# Autodesk Inventor assembly: 机械架构
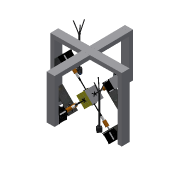
[picture p0: Inventor's stored thumbnail of the model, 180x180]
Saved by Autodesk Inventor 2016 (Build 200138000, 138)
## iProperties
Created: 2019-05-19
Part Number: 机械架构
Material: 常规
Document SubType Name: Assembly
Designer: oldboy
Author: oldboy
## Documents named in this file (14)
- F:\folder\毕业设计\解魔方机器人\机械结构\机械架构.iam
- F:\folder\毕业设计\解魔方机器人\机械结构\步进电机.ipt
- F:\folder\毕业设计\解魔方机器人\机械结构\杆件.ipt
- F:\folder\毕业设计\解魔方机器人\机械结构\联轴器.ipt
- F:\folder\毕业设计\解魔方机器人\机械结构\机械爪六角筒.ipt
- F:\folder\毕业设计\解魔方机器人\机械结构\机械架构\设计加速器\压缩弹簧1.iam
- F:\folder\毕业设计\解魔方机器人\机械结构\螺母.ipt
- F:\folder\毕业设计\解魔方机器人\机械结构\欧标铝.ipt
- F:\folder\毕业设计\解魔方机器人\机械结构\45度角件.ipt
- F:\folder\毕业设计\解魔方机器人\机械结构\魔方.ipt
- F:\folder\毕业设计\解魔方机器人\机械结构\欧标铝-354.299mm.ipt
- F:\folder\毕业设计\解魔方机器人\机械结构\欧标铝-221.402mm.ipt
- F:\folder\毕业设计\解魔方机器人\机械结构\欧标铝-180mm.ipt
- F:\folder\毕业设计\解魔方机器人\机械结构\摄像头.ipt
## Components (50 placed, 13 different names)
1. 步进电机:5 — 插入:1, 插入:4, 表面齐平:4
2. 联轴器:1 — 插入:1, 插入:3
3. 机械爪六角筒:1 — 配合:2, 圆柱:1, 插入:3
4. 杆件:1 — 配合:1, 表面齐平:1, 圆柱:1, 插入:2, 插入:9
5. 压缩弹簧:1 [sub-assembly] — 配合:1, 表面齐平:1, 配合:2
6. 螺母:1 — 插入:2
7. 45度角件:1 — 插入:4, 表面齐平:4, 配合:5, 表面齐平:7, 表面齐平:8
8. 魔方:1 — 插入:9, 插入:14, 插入:15, 插入:24, 插入:25, 插入:26, 插入:27, 插入:31, 插入:32, 插入:36, 插入:37
9. 步进电机:6
10. 联轴器:2
11. 机械爪六角筒:2
12. 杆件:2 — 插入:14, 插入:15
13. 压缩弹簧:2 [sub-assembly]
14. 螺母:2
15. 45度角件:2 — 表面齐平:9
16. 欧标铝:1 — 配合:5, 表面齐平:7, 表面齐平:8, 表面齐平:9, 表面齐平:17, 表面齐平:23, 配合:16, 表面齐平:28
17. 步进电机:7
18. 联轴器:3
19. 机械爪六角筒:3
20. 杆件:3 — 插入:24, 插入:25
21. 压缩弹簧:3 [sub-assembly]
22. 螺母:3
23. 45度角件:3
24. 步进电机:8
25. 联轴器:4
26. 机械爪六角筒:4
27. 杆件:4 — 插入:26, 插入:27
28. 压缩弹簧:4 [sub-assembly]
29. 螺母:4
30. 45度角件:4
31. 欧标铝:2 — 表面齐平:17
32. 步进电机:9 — 配合:17, 表面齐平:25
33. 联轴器:5
34. 机械爪六角筒:5
35. 杆件:5 — 插入:31, 插入:32
36. 压缩弹簧:5 [sub-assembly]
37. 螺母:5
38. 步进电机:10 — 配合:19, 表面齐平:30
39. 联轴器:6
40. 机械爪六角筒:6
41. 杆件:6 — 插入:36, 插入:37
42. 压缩弹簧:6 [sub-assembly]
43. 螺母:6
44. 欧标铝-221.402mm:1 — 配合:19, 表面齐平:29, 表面齐平:30, 表面齐平:32, 角度:2
45. 欧标铝-221.402mm:2 — 配合:17, 表面齐平:24, 表面齐平:25, 表面齐平:27, 表面齐平:33, 角度:1
46. 欧标铝-354.299mm:1 — 表面齐平:23, 配合:16, 表面齐平:24, 表面齐平:26, 配合:18, 表面齐平:28, 表面齐平:29, 配合:20, 表面齐平:31
47. 欧标铝-180mm:1 — 表面齐平:26, 配合:18, 表面齐平:27
48. 欧标铝-180mm:2 — 配合:20, 表面齐平:31, 表面齐平:32, 表面齐平:34, 表面齐平:35
49. 摄像头:1 — 表面齐平:33, 角度:1
50. 摄像头:2 — 表面齐平:34, 角度:2
## Relationships (90: Insert 33, Flush 30, Mate 19, CylindricalJoint 6, Angle 2)
- 插入:1 [Insert] (-10 mm): 步进电机:5 ↔ 联轴器:1
- 配合:1 [Mate]: 杆件:1 ↔ 压缩弹簧:1
- 表面齐平:1 [Flush]: 杆件:1 ↔ 压缩弹簧:1
- 配合:2 [Mate]: 机械爪六角筒:1 ↔ 压缩弹簧:1
- 圆柱:1 [CylindricalJoint]: 机械爪六角筒:1 ↔ 杆件:1
- 插入:2 [Insert] (-2 mm): 杆件:1 ↔ 螺母:1
- 插入:3 [Insert] (-6 mm): 联轴器:1 ↔ 机械爪六角筒:1
- 插入:4 [Insert]: 步进电机:5 ↔ 45度角件:1
- 表面齐平:4 [Flush]: 步进电机:5 ↔ 45度角件:1
- 插入:9 [Insert] (-4.5 mm): 杆件:1 ↔ 魔方:1
- [Insert] (-10 mm): 步进电机:6 ↔ 联轴器:2
- [Mate]: 杆件:2 ↔ 压缩弹簧:2
- [Flush]: 杆件:2 ↔ 压缩弹簧:2
- [Mate]: 机械爪六角筒:2 ↔ 压缩弹簧:2
- [CylindricalJoint]: 机械爪六角筒:2 ↔ 杆件:2
- [Insert] (-2 mm): 杆件:2 ↔ 螺母:2
- [Insert] (-6 mm): 联轴器:2 ↔ 机械爪六角筒:2
- [Insert]: 步进电机:6 ↔ 45度角件:2
- [Flush]: 步进电机:6 ↔ 45度角件:2
- 插入:14 [Insert] (-4.5 mm): 魔方:1 ↔ 杆件:2
- 插入:15 [Insert] (-4.5 mm): 魔方:1 ↔ 杆件:2
- 配合:5 [Mate]: 45度角件:1 ↔ 欧标铝:1
- 表面齐平:7 [Flush] (-1 mm): 45度角件:1 ↔ 欧标铝:1
- 表面齐平:8 [Flush] (20 mm): 45度角件:1 ↔ 欧标铝:1
- 表面齐平:9 [Flush] (-1 mm): 45度角件:2 ↔ 欧标铝:1
- [Insert] (-10 mm): 步进电机:7 ↔ 联轴器:3
- [Mate]: 杆件:3 ↔ 压缩弹簧:3
- [Flush]: 杆件:3 ↔ 压缩弹簧:3
- [Mate]: 机械爪六角筒:3 ↔ 压缩弹簧:3
- [CylindricalJoint]: 机械爪六角筒:3 ↔ 杆件:3
- [Insert] (-2 mm): 杆件:3 ↔ 螺母:3
- [Insert] (-6 mm): 联轴器:3 ↔ 机械爪六角筒:3
- [Insert]: 步进电机:7 ↔ 45度角件:3
- [Flush]: 步进电机:7 ↔ 45度角件:3
- [Insert] (-10 mm): 步进电机:8 ↔ 联轴器:4
- [Mate]: 杆件:4 ↔ 压缩弹簧:4
- [Flush]: 杆件:4 ↔ 压缩弹簧:4
- [Mate]: 机械爪六角筒:4 ↔ 压缩弹簧:4
- [CylindricalJoint]: 机械爪六角筒:4 ↔ 杆件:4
- [Insert] (-2 mm): 杆件:4 ↔ 螺母:4
- [Insert] (-6 mm): 联轴器:4 ↔ 机械爪六角筒:4
- [Insert]: 步进电机:8 ↔ 45度角件:4
- [Flush]: 步进电机:8 ↔ 45度角件:4
- [Mate]: 45度角件:3 ↔ 欧标铝:2
- [Flush] (-1 mm): 45度角件:3 ↔ 欧标铝:2
- [Flush] (20 mm): 45度角件:3 ↔ 欧标铝:2
- [Flush] (-1 mm): 45度角件:4 ↔ 欧标铝:2
- 插入:24 [Insert] (0.5 mm): 魔方:1 ↔ 杆件:3
- 插入:25 [Insert] (0.5 mm): 魔方:1 ↔ 杆件:3
- 表面齐平:17 [Flush]: 欧标铝:1 ↔ 欧标铝:2
- 插入:26 [Insert] (-4.5 mm): 魔方:1 ↔ 杆件:4
- 插入:27 [Insert] (-4.5 mm): 魔方:1 ↔ 杆件:4
- [Insert] (-10 mm): 步进电机:9 ↔ 联轴器:5
- [Mate]: 杆件:5 ↔ 压缩弹簧:5
- [Flush]: 杆件:5 ↔ 压缩弹簧:5
- [Mate]: 机械爪六角筒:5 ↔ 压缩弹簧:5
- [CylindricalJoint]: 机械爪六角筒:5 ↔ 杆件:5
- [Insert] (-2 mm): 杆件:5 ↔ 螺母:5
- [Insert] (-6 mm): 联轴器:5 ↔ 机械爪六角筒:5
- 插入:31 [Insert] (-0.5 mm): 魔方:1 ↔ 杆件:5
- 插入:32 [Insert] (0.5 mm): 魔方:1 ↔ 杆件:5
- [Insert] (-10 mm): 步进电机:10 ↔ 联轴器:6
- [Mate]: 杆件:6 ↔ 压缩弹簧:6
- [Flush]: 杆件:6 ↔ 压缩弹簧:6
- [Mate]: 机械爪六角筒:6 ↔ 压缩弹簧:6
- [CylindricalJoint]: 机械爪六角筒:6 ↔ 杆件:6
- [Insert] (-2 mm): 杆件:6 ↔ 螺母:6
- [Insert] (-6 mm): 联轴器:6 ↔ 机械爪六角筒:6
- 插入:36 [Insert] (-4.5 mm): 魔方:1 ↔ 杆件:6
- 插入:37 [Insert] (-4.5 mm): 魔方:1 ↔ 杆件:6
- 表面齐平:23 [Flush]: 欧标铝:1 ↔ 欧标铝-354.299mm:1
- 配合:16 [Mate]: 欧标铝:1 ↔ 欧标铝-354.299mm:1
- 配合:17 [Mate]: 步进电机:9 ↔ 欧标铝-221.402mm:2
- 表面齐平:24 [Flush]: 欧标铝-221.402mm:2 ↔ 欧标铝-354.299mm:1
- 表面齐平:25 [Flush]: 步进电机:9 ↔ 欧标铝-221.402mm:2
- 表面齐平:26 [Flush]: 欧标铝-354.299mm:1 ↔ 欧标铝-180mm:1
- 配合:18 [Mate]: 欧标铝-354.299mm:1 ↔ 欧标铝-180mm:1
- 表面齐平:27 [Flush]: 欧标铝-221.402mm:2 ↔ 欧标铝-180mm:1
- 表面齐平:28 [Flush]: 欧标铝:1 ↔ 欧标铝-354.299mm:1
- 配合:19 [Mate]: 步进电机:10 ↔ 欧标铝-221.402mm:1
- 表面齐平:29 [Flush]: 欧标铝-221.402mm:1 ↔ 欧标铝-354.299mm:1
- 表面齐平:30 [Flush]: 步进电机:10 ↔ 欧标铝-221.402mm:1
- 配合:20 [Mate]: 欧标铝-354.299mm:1 ↔ 欧标铝-180mm:2
- 表面齐平:31 [Flush]: 欧标铝-354.299mm:1 ↔ 欧标铝-180mm:2
- 表面齐平:32 [Flush]: 欧标铝-221.402mm:1 ↔ 欧标铝-180mm:2
- 表面齐平:33 [Flush]: 欧标铝-221.402mm:2 ↔ 摄像头:1
- 角度:1 [Angle] (126 deg): 欧标铝-221.402mm:2 ↔ 摄像头:1
- 表面齐平:34 [Flush]: 欧标铝-180mm:2 ↔ 摄像头:2
- 角度:2 [Angle] (126 deg): 欧标铝-221.402mm:1 ↔ 摄像头:2
- 表面齐平:35 [Flush]: 欧标铝-180mm:2
## Named parameters: d82_d78 = 0 mm, d83_d33 = -2 mm, d84_d40 = -6 mm, d85_d43 = 0 mm, d86_d8 = -37.700105 deg, d87_d9 = 1.99999 mm, d88_d3 = -10 mm, d89_d5 = 0 mm, d90_d6 = 0 mm, d91_d7 = 0 mm, d122_d120 = 20 mm, d123_d121 = -1 mm, d124_d118 = 0 mm, d125_d119 = -1 mm, d126_d78 = 0 mm, d127_d82_d78 = 0 mm, d128_d83_d33 = -2 mm, d129_d84_d40 = -6 mm, d130_d85_d43 = 0 mm, d131_d86_d8 = -122.773065 deg, d132_d87_d9 = 1.99999 mm, d133_d88_d3 = -10 mm, d134_d89_d5 = 0 mm, d135_d90_d6 = 0 mm, d136_d91_d7 = 0 mm, d137_d33 = -2 mm, d138_d40 = -6 mm, d139_d43 = 0 mm, d140_d8 = 50.13186 deg, d141_d9 = 1.99999 mm, d142_d3 = -10 mm, d143_d5 = 0 mm, d144_d6 = 0 mm, d145_d7 = 0 mm, d203_d33 = -2 mm, d204_d40 = -6 mm, d206_d8 = 137.620954 deg, d207_d9 = 1.99999 mm, d208_d3 = -10 mm, d209_d5 = 0 mm, d210_d6 = 0 mm, d211_d7 = 0 mm, d239_d33 = -2 mm, d240_d40 = -6 mm, d242_d8 = -162.306166 deg, d243_d9 = 1.99999 mm, d244_d3 = -10 mm, d245_d5 = 0 mm, d246_d6 = 0 mm, d247_d7 = 0 mm
